# Autodesk Inventor assembly: Assembly11
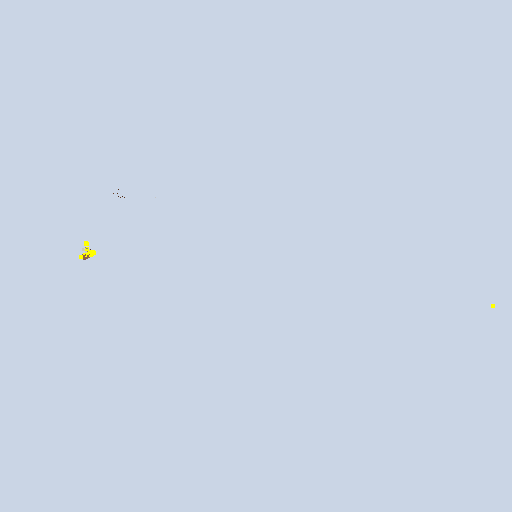
[picture p0: Inventor's stored thumbnail of the model, 512x512]
Saved by Autodesk Inventor 2024.1 (Build 281209000, 209)
## iProperties
Created: 2023-11-10
Part Number: Assembly11
Document SubType Name: Assembly
Designer: luvag
Author: luvag
## Documents named in this file (3)
- C:\Users\luvag\Desktop\Assembly11.iam
- C:\Users\luvag\Desktop\Assembly23.iam
- C:\Users\luvag\Desktop\Maitri_chair.ipt
## Components (2 placed, 2 different names)
1. Assembly23:1 [sub-assembly]
2. Maitri_chair:1
## Relationships (1: Mate 1)
- [Mate] (254 mm): Assembly23:1 ↔ Maitri_chair:1
